# Autodesk Inventor assembly: bracepost
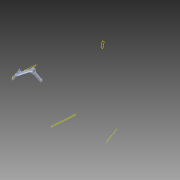
[picture p0: Inventor's stored thumbnail of the model, 180x180]
Saved by Autodesk Inventor 2014 SP1 (Build 180222100, 222)
## iProperties
Created: 2014-01-05
Part Number: bracepost
Document SubType Name: Assembly
Designer: Andrew Toennies
Mass: 236.023 g
Surface Area: 1461.88 cm^2
Volume: 117.734 cm^3
Density: 2.00471 g/cm^3
Author: Andrew Toennies
## Documents named in this file (8)
- C:\Users\Arpan\Documents\GitHub\2014buildCAD\Shooter\bracepost.iam
- C:\Users\Arpan\Documents\GitHub\2014buildCAD\Shooter\Vex Pro 1x1 rectangular tubing 12 in length.ipt
- C:\Users\Arpan\Documents\GitHub\2014buildCAD\Shooter\Vex Pro Corner Gusset.ipt
- C:\Users\Arpan\Documents\GitHub\2014buildCAD\Shooter\Vex Pro Side Bearing Gusset.ipt
- C:\Users\Arpan\Documents\GitHub\2014buildCAD\Shooter\Bearing ID 0.375 OD 1.125.ipt
- C:\Users\Arpan\Documents\GitHub\2014buildCAD\Shooter\Vex Pro 30 tooth 9mm timing belt pulley.ipt
- C:\Users\Arpan\Documents\GitHub\2014buildCAD\Shooter\armbackspacer.ipt
- C:\Users\Arpan\Documents\GitHub\2014buildCAD\Shooter\Vex Pro 1x1 rectangular tubing 6  in length chamfered.ipt
## Components (11 placed, 7 different names)
1. Vex Pro 1x1 rectangular tubing 12 in length:1 — Insert:9, Insert:10, Insert:11, Insert:12, Flush:4, Mate:23, Mate:24, Mate:25, Mate:26, Mate:27, Mate:28, Flush:15
2. Vex Pro Corner Gusset:1 — Insert:9, Insert:10
3. Vex Pro Corner Gusset:2 — Insert:11, Insert:12
4. Vex Pro 30 tooth 9mm timing belt pulley:1
5. armbackspacer:1 — Mate:26, Mate:27, Mate:28, Mate:29, Mate:30, Mate:31
6. armbackspacer:2 — Mate:23, Mate:24, Mate:25, Mate:32, Flush:13, Flush:14
7. Vex Pro Side Bearing Gusset:1 — Mate:29, Mate:30, Mate:31, Mate:33
8. Vex Pro Side Bearing Gusset:2 — Mate:32, Flush:13, Flush:14, Mate:34
9. Bearing ID 0.375 OD 1.125:1 — Mate:34, Mate:35
10. Bearing ID 0.375 OD 1.125:2 — Mate:33
11. Vex Pro 1x1 rectangular tubing 6  in length chamfered:1 — Mate:35, Flush:15
## Relationships (22: Mate 13, Flush 5, Insert 4)
- Insert:9: Vex Pro 1x1 rectangular tubing 12 in length:1 ↔ Vex Pro Corner Gusset:1
- Insert:10: Vex Pro 1x1 rectangular tubing 12 in length:1 ↔ Vex Pro Corner Gusset:1
- Insert:11: Vex Pro 1x1 rectangular tubing 12 in length:1 ↔ Vex Pro Corner Gusset:2
- Insert:12: Vex Pro 1x1 rectangular tubing 12 in length:1 ↔ Vex Pro Corner Gusset:2
- Flush:4: Vex Pro 1x1 rectangular tubing 12 in length:1
- Flush:5 (-711.2 mm)
- Mate:23: Vex Pro 1x1 rectangular tubing 12 in length:1 ↔ armbackspacer:2
- Mate:24: Vex Pro 1x1 rectangular tubing 12 in length:1 ↔ armbackspacer:2
- Mate:25: Vex Pro 1x1 rectangular tubing 12 in length:1 ↔ armbackspacer:2
- Mate:26: Vex Pro 1x1 rectangular tubing 12 in length:1 ↔ armbackspacer:1
- Mate:27: Vex Pro 1x1 rectangular tubing 12 in length:1 ↔ armbackspacer:1
- Mate:28: Vex Pro 1x1 rectangular tubing 12 in length:1 ↔ armbackspacer:1
- Mate:29: armbackspacer:1 ↔ Vex Pro Side Bearing Gusset:1
- Mate:30: armbackspacer:1 ↔ Vex Pro Side Bearing Gusset:1
- Mate:31: armbackspacer:1 ↔ Vex Pro Side Bearing Gusset:1
- Mate:32: armbackspacer:2 ↔ Vex Pro Side Bearing Gusset:2
- Flush:13: armbackspacer:2 ↔ Vex Pro Side Bearing Gusset:2
- Flush:14: armbackspacer:2 ↔ Vex Pro Side Bearing Gusset:2
- Mate:33: Vex Pro Side Bearing Gusset:1 ↔ Bearing ID 0.375 OD 1.125:2
- Mate:34: Vex Pro Side Bearing Gusset:2 ↔ Bearing ID 0.375 OD 1.125:1
- Mate:35: Bearing ID 0.375 OD 1.125:1 ↔ Vex Pro 1x1 rectangular tubing 6  in length chamfered:1
- Flush:15: Vex Pro 1x1 rectangular tubing 12 in length:1 ↔ Vex Pro 1x1 rectangular tubing 6  in length chamfered:1
